# Autodesk Inventor assembly: 2024-210-Fixed-Shootaur
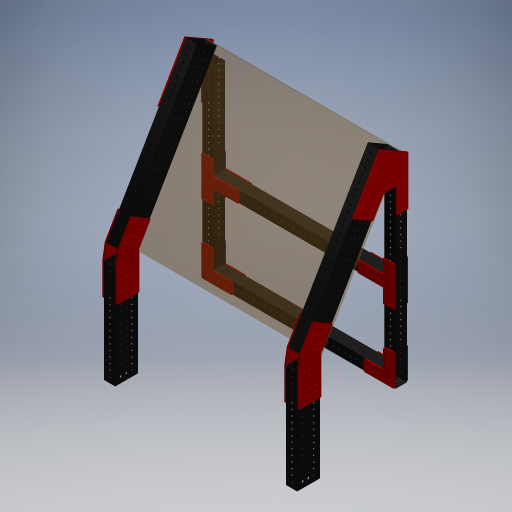
[picture p0: Inventor's stored thumbnail of the model, 512x512]
Saved by Autodesk Inventor 2024.2 (Build 282272000, 272)
## iProperties
Created: 2024-02-11
Part Number: 2024-210-Fixed-Shootaur
Document SubType Name: Assembly
Designer: rohan
Author: rohan
## Documents named in this file (11)
- C:\Users\rohan\OneDrive - Hillsborough County Public Schools\Robotics\FIRST-Robotics-Competition\Crescendo\Minotaur-Crescendo-Robot\Structure\Superstructure\Fixed Shooter\2024-210-Fixed-Shootaur.iam
- C:\Users\rohan\OneDrive - Hillsborough County Public Schools\Robotics\FIRST-Robotics-Competition\Crescendo\Minotaur-Crescendo-Robot\Structure\Superstructure\Fixed Shooter\2024-210-004-Back-Gusset.ipt
- C:\Users\rohan\OneDrive - Hillsborough County Public Schools\Robotics\FIRST-Robotics-Competition\Crescendo\Minotaur-Crescendo-Robot\Structure\Superstructure\Fixed Shooter\2024-210-005-Front-Gusset.ipt
- C:\Users\rohan\OneDrive - Hillsborough County Public Schools\Robotics\FIRST-Robotics-Competition\Crescendo\Minotaur-Crescendo-Robot\Structure\Superstructure\Fixed Shooter\2024-210-001-Shooter-Beam.ipt
- C:\Users\rohan\OneDrive - Hillsborough County Public Schools\Robotics\FIRST-Robotics-Competition\Crescendo\Minotaur-Crescendo-Robot\Structure\Superstructure\Fixed Shooter\2024-210-003-Front-Angle.ipt
- C:\Users\rohan\OneDrive - Hillsborough County Public Schools\Robotics\FIRST-Robotics-Competition\Crescendo\Minotaur-Crescendo-Robot\Structure\Superstructure\Fixed Shooter\2024-210-002-Backright-Support.ipt
- C:\Users\rohan\OneDrive - Hillsborough County Public Schools\Robotics\FIRST-Robotics-Competition\Crescendo\Minotaur-Crescendo-Robot\Structure\Superstructure\Fixed Shooter\2024-210-006-Underside-Mount.ipt
- C:\Users\rohan\OneDrive - Hillsborough County Public Schools\Robotics\FIRST-Robotics-Competition\Crescendo\Minotaur-Crescendo-Robot\Structure\Superstructure\Fixed Shooter\2024-210-007-Left-Right-Support.ipt
- C:\Users\rohan\OneDrive - Hillsborough County Public Schools\Robotics\FIRST-Robotics-Competition\Crescendo\Minotaur-Crescendo-Robot\Structure\Gussets\THRIFYBOT-L-Gusset.ipt
- C:\Users\rohan\OneDrive - Hillsborough County Public Schools\Robotics\FIRST-Robotics-Competition\Crescendo\Minotaur-Crescendo-Robot\Structure\Gussets\THRIFYBOT-T-Gusset.ipt
- C:\Users\rohan\OneDrive - Hillsborough County Public Schools\Robotics\FIRST-Robotics-Competition\Crescendo\Minotaur-Crescendo-Robot\Structure\Superstructure\Polycarbonate-Note-Rest.ipt
## Components (23 placed, 10 different names)
1. 2024-210-004-Back-Gusset:1 — Flush:1, Flush:2, Mate:1, Flush:9
2. 2024-210-004-Back-Gusset:2 — Flush:1, Flush:2, Mate:1, Mate:3, Flush:5, Insert:1, Mate:6, Insert:3
3. 2024-210-005-Front-Gusset:2 — Flush:23, Mate:22, Flush:24, Mate:25, Flush:26, Mate:26
4. 2024-210-001-Shooter-Beam:1 — Mate:3, Flush:5, Insert:1, Flush:23, Mate:22, Flush:24, Mate:37, Flush:46, Flush:47
5. 2024-210-002-Backright-Support:1 — Mate:6, Flush:9, Insert:3, Flush:19, Flush:20, Mate:13
6. 2024-210-004-Back-Gusset:3
7. 2024-210-004-Back-Gusset:4
8. 2024-210-005-Front-Gusset:3 — Mate:21, Flush:21, Flush:22, Mate:23, Flush:25, Mate:24
9. 2024-210-001-Shooter-Beam:2 — Mate:21, Flush:21, Flush:22
10. 2024-210-002-Backright-Support:2 — Flush:19, Flush:20, Mate:13
11. 2024-210-003-Front-Angle:1 — Mate:25, Flush:26, Mate:26, Mate:27, Mate:28, Flush:34, Insert:8, Mate:36, Flush:44
12. 2024-210-003-Front-Angle:2 — Mate:23, Flush:25, Mate:24, Flush:27, Flush:28, Flush:29, Flush:36, Mate:32, Insert:7, Mate:35, Flush:43
13. 2024-210-006-Underside-Mount:1 — Mate:27, Flush:27, Flush:28, Mate:31, Flush:35, Flush:37
14. 2024-210-007-Left-Right-Support:1 — Mate:28, Flush:29, Flush:42, Flush:45
15. THRIFYBOT-L-Gusset:1 — Flush:30, Flush:31, Mate:29
16. THRIFYBOT-L-Gusset:2 — Flush:30, Flush:31, Mate:29, Mate:31, Flush:34, Flush:35, Insert:8
17. THRIFYBOT-L-Gusset:3 — Flush:36, Insert:7
18. THRIFYBOT-L-Gusset:4 — Mate:32, Flush:37
19. THRIFYBOT-T-Gusset:1 — Flush:38, Flush:39, Mate:33, Mate:35, Flush:42, Flush:43
20. THRIFYBOT-T-Gusset:2 — Flush:38, Flush:39, Mate:33
21. THRIFYBOT-T-Gusset:3 — Mate:36, Flush:44, Flush:45
22. THRIFYBOT-T-Gusset:4
23. Polycarbonate-Note-Rest:1 — Mate:37, Flush:46, Flush:47
## Relationships (67: Flush 37, Mate 24, Insert 6)
- Flush:1: 2024-210-004-Back-Gusset:1 ↔ 2024-210-004-Back-Gusset:2
- Flush:2: 2024-210-004-Back-Gusset:1 ↔ 2024-210-004-Back-Gusset:2
- Mate:1 (25.4 mm): 2024-210-004-Back-Gusset:1 ↔ 2024-210-004-Back-Gusset:2
- Mate:3: 2024-210-004-Back-Gusset:2 ↔ 2024-210-001-Shooter-Beam:1
- Flush:5: 2024-210-004-Back-Gusset:2 ↔ 2024-210-001-Shooter-Beam:1
- Insert:1: 2024-210-004-Back-Gusset:2 ↔ 2024-210-001-Shooter-Beam:1
- Mate:6: 2024-210-004-Back-Gusset:2 ↔ 2024-210-002-Backright-Support:1
- Flush:9: 2024-210-004-Back-Gusset:1 ↔ 2024-210-002-Backright-Support:1
- Insert:3: 2024-210-004-Back-Gusset:2 ↔ 2024-210-002-Backright-Support:1
- [Flush]: 2024-210-004-Back-Gusset:3 ↔ 2024-210-004-Back-Gusset:4
- [Flush]: 2024-210-004-Back-Gusset:3 ↔ 2024-210-004-Back-Gusset:4
- [Mate] (25.4 mm): 2024-210-004-Back-Gusset:3 ↔ 2024-210-004-Back-Gusset:4
- [Mate]: 2024-210-004-Back-Gusset:4 ↔ 2024-210-001-Shooter-Beam:2
- [Flush]: 2024-210-004-Back-Gusset:4 ↔ 2024-210-001-Shooter-Beam:2
- [Insert]: 2024-210-004-Back-Gusset:4 ↔ 2024-210-001-Shooter-Beam:2
- [Mate]: 2024-210-004-Back-Gusset:4 ↔ 2024-210-002-Backright-Support:2
- [Flush]: 2024-210-004-Back-Gusset:3 ↔ 2024-210-002-Backright-Support:2
- [Insert]: 2024-210-004-Back-Gusset:4 ↔ 2024-210-002-Backright-Support:2
- Flush:19: 2024-210-002-Backright-Support:1 ↔ 2024-210-002-Backright-Support:2
- Flush:20: 2024-210-002-Backright-Support:1 ↔ 2024-210-002-Backright-Support:2
- Mate:13 (381 mm): 2024-210-002-Backright-Support:1 ↔ 2024-210-002-Backright-Support:2
- Mate:21: 2024-210-005-Front-Gusset:3 ↔ 2024-210-001-Shooter-Beam:2
- Flush:21: 2024-210-005-Front-Gusset:3 ↔ 2024-210-001-Shooter-Beam:2
- Flush:22: 2024-210-005-Front-Gusset:3 ↔ 2024-210-001-Shooter-Beam:2
- Flush:23: 2024-210-005-Front-Gusset:2 ↔ 2024-210-001-Shooter-Beam:1
- Mate:22: 2024-210-005-Front-Gusset:2 ↔ 2024-210-001-Shooter-Beam:1
- Flush:24: 2024-210-005-Front-Gusset:2 ↔ 2024-210-001-Shooter-Beam:1
- Mate:23: 2024-210-005-Front-Gusset:3 ↔ 2024-210-003-Front-Angle:2
- Flush:25: 2024-210-005-Front-Gusset:3 ↔ 2024-210-003-Front-Angle:2
- Mate:24: 2024-210-005-Front-Gusset:3 ↔ 2024-210-003-Front-Angle:2
- Mate:25: 2024-210-005-Front-Gusset:2 ↔ 2024-210-003-Front-Angle:1
- Flush:26: 2024-210-005-Front-Gusset:2 ↔ 2024-210-003-Front-Angle:1
- Mate:26: 2024-210-005-Front-Gusset:2 ↔ 2024-210-003-Front-Angle:1
- Mate:27: 2024-210-003-Front-Angle:1 ↔ 2024-210-006-Underside-Mount:1
- Flush:27: 2024-210-003-Front-Angle:2 ↔ 2024-210-006-Underside-Mount:1
- Flush:28: 2024-210-003-Front-Angle:2 ↔ 2024-210-006-Underside-Mount:1
- Mate:28: 2024-210-003-Front-Angle:1 ↔ 2024-210-007-Left-Right-Support:1
- Flush:29: 2024-210-003-Front-Angle:2 ↔ 2024-210-007-Left-Right-Support:1
- Flush:30: THRIFYBOT-L-Gusset:1 ↔ THRIFYBOT-L-Gusset:2
- Flush:31: THRIFYBOT-L-Gusset:1 ↔ THRIFYBOT-L-Gusset:2
- Mate:29 (25.4 mm): THRIFYBOT-L-Gusset:1 ↔ THRIFYBOT-L-Gusset:2
- [Flush]: THRIFYBOT-L-Gusset:3 ↔ THRIFYBOT-L-Gusset:4
- [Flush]: THRIFYBOT-L-Gusset:3 ↔ THRIFYBOT-L-Gusset:4
- [Mate] (25.4 mm): THRIFYBOT-L-Gusset:3 ↔ THRIFYBOT-L-Gusset:4
- Mate:31: 2024-210-006-Underside-Mount:1 ↔ THRIFYBOT-L-Gusset:2
- Flush:34: 2024-210-003-Front-Angle:1 ↔ THRIFYBOT-L-Gusset:2
- Flush:35: 2024-210-006-Underside-Mount:1 ↔ THRIFYBOT-L-Gusset:2
- Flush:36: 2024-210-003-Front-Angle:2 ↔ THRIFYBOT-L-Gusset:3
- Mate:32: 2024-210-003-Front-Angle:2 ↔ THRIFYBOT-L-Gusset:4
- Flush:37: 2024-210-006-Underside-Mount:1 ↔ THRIFYBOT-L-Gusset:4
- Insert:7: 2024-210-003-Front-Angle:2 ↔ THRIFYBOT-L-Gusset:3
- Insert:8: 2024-210-003-Front-Angle:1 ↔ THRIFYBOT-L-Gusset:2
- Flush:38: THRIFYBOT-T-Gusset:1 ↔ THRIFYBOT-T-Gusset:2
- Flush:39: THRIFYBOT-T-Gusset:1 ↔ THRIFYBOT-T-Gusset:2
- Mate:33 (25.4 mm): THRIFYBOT-T-Gusset:1 ↔ THRIFYBOT-T-Gusset:2
- [Flush]: THRIFYBOT-T-Gusset:3 ↔ THRIFYBOT-T-Gusset:4
- [Flush]: THRIFYBOT-T-Gusset:3 ↔ THRIFYBOT-T-Gusset:4
- [Mate] (25.4 mm): THRIFYBOT-T-Gusset:3 ↔ THRIFYBOT-T-Gusset:4
- Mate:35: 2024-210-003-Front-Angle:2 ↔ THRIFYBOT-T-Gusset:1
- Flush:42: 2024-210-007-Left-Right-Support:1 ↔ THRIFYBOT-T-Gusset:1
- Flush:43: 2024-210-003-Front-Angle:2 ↔ THRIFYBOT-T-Gusset:1
- Mate:36: 2024-210-003-Front-Angle:1 ↔ THRIFYBOT-T-Gusset:3
- Flush:44: 2024-210-003-Front-Angle:1 ↔ THRIFYBOT-T-Gusset:3
- Flush:45: 2024-210-007-Left-Right-Support:1 ↔ THRIFYBOT-T-Gusset:3
- Mate:37: 2024-210-001-Shooter-Beam:1 ↔ Polycarbonate-Note-Rest:1
- Flush:46: 2024-210-001-Shooter-Beam:1 ↔ Polycarbonate-Note-Rest:1
- Flush:47: 2024-210-001-Shooter-Beam:1 ↔ Polycarbonate-Note-Rest:1
## Named parameters: d18_d0 = 0 mm, d19_d1 = 0 mm, d20_d2 = 25.4 mm, d24_d6 = 0 mm, d25_d7 = 0 mm, d26_d8 = 0 mm, d33_d15 = 0 mm, d34_d16 = 0 mm, d35_d17 = 0 mm, d75_d72 = 0 mm, d76_d73 = 0 mm, d77_d74 = 25.4 mm, d89_d86 = 0 mm, d90_d87 = 0 mm, d91_d88 = 25.4 mm
